# Autodesk Inventor assembly: Unwrap_wing
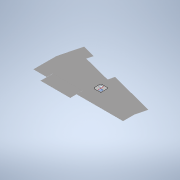
[picture p0: Inventor's stored thumbnail of the model, 180x180]
Saved by Autodesk Inventor 2020 (Build 240168000, 168)
## iProperties
Created: 2020-03-08
Part Number: Unwrap_wing
Document SubType Name: Assembly
Designer: valem
Author: valem
## Documents named in this file (3)
- D:\Planes\Cardboard_glider_1\Unwrap_wing.iam
- D:\Planes\Cardboard_glider_1\unwrap_wing.ipt
- D:\Planes\Cardboard_glider_1\unwrap_aileron.ipt
## Components (2 placed, 2 different names)
1. unwrap_wing:1 — Mate:1, Mate:3, Mate:4
2. unwrap_aileron:1 — Mate:2, Mate:4
## Relationships (4: Mate 4)
- Mate:1: unwrap_wing:1
- Mate:2: unwrap_aileron:1
- Mate:3: unwrap_wing:1
- Mate:4 (0.5 mm): unwrap_wing:1 ↔ unwrap_aileron:1
